# Autodesk Inventor assembly: main
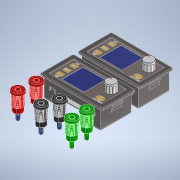
[picture p0: Inventor's stored thumbnail of the model, 180x180]
Saved by Autodesk Inventor 2022.1 (Build 261234020, 234B)
## iProperties
Created: 2022-02-06
Part Number: main
Document SubType Name: Assembly
Designer: kee
Mass: 95.8052 g
Surface Area: 852.993 cm^2
Volume: 46.3616 cm^3
Density: 2.06648 g/cm^3
Author: kee
## Documents named in this file (3)
- C:\Users\logic\_workspace\2-ch-power-supply\hardware\casing\main.iam
- C:\Users\logic\_workspace\2-ch-power-supply\hardware\casing\standard_parts\DPS-5015\DPS_5015.iam
- C:\Users\logic\_workspace\2-ch-power-supply\hardware\casing\standard_parts\banana_jack\CT2236-0.iam
## Components (8 placed, 3 different names)
1. DPS_5015:1 [sub-assembly] — Flush:1, Flush:2, Mate:1, Flush:3
2. DPS_5015:2 [sub-assembly] — Flush:1, Flush:2, Mate:1, Mate:2
3. CT2236-black:1 [sub-assembly] — Flush:4
4. CT2236-0:2 [sub-assembly]
5. CT2236-0:3 [sub-assembly]
6. CT2236-0:5 [sub-assembly] — Mate:2
7. CT2236-0:6 [sub-assembly]
8. CT2236-0:7 [sub-assembly]
## Relationships (6: Flush 4, Mate 2)
- Flush:1: DPS_5015:1 ↔ DPS_5015:2
- Flush:2: DPS_5015:1 ↔ DPS_5015:2
- Mate:1 (5 mm): DPS_5015:1 ↔ DPS_5015:2
- Flush:3: DPS_5015:1
- Flush:4: CT2236-black:1
- Mate:2: DPS_5015:2 ↔ CT2236-0:5
